# Autodesk Inventor assembly: Moving_Link_Fixation
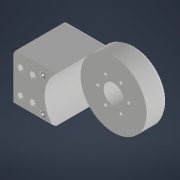
[picture p0: Inventor's stored thumbnail of the model, 180x180]
Saved by Autodesk Inventor 2021 (Build 250183000, 183)
## iProperties
Created: 2025-04-04
Part Number: Moving_Link_Fixation
Document SubType Name: Assembly
Designer: rocke
Author: rocke
## Documents named in this file (5)
- C:\Users\rocke\Documents\Robot Arm IPT\Moving Link Fixation\Moving_Link_Fixation.iam
- C:\Users\rocke\Documents\Inventor\Content Center Files\R2021\en-US\ISO 4032(2)\ISO 4032 - M4 - ISO.ipt
- C:\Users\rocke\Documents\Inventor\Content Center Files\R2021\en-US\ANSI B18.3.1M(1)\ANSI B18.3.1M - M4x0.7 x 65(2).ipt
- C:\Users\rocke\Documents\Robot Arm IPT\Moving Link Fixation\Moving_Link_Fixation_Small.ipt
- C:\Users\rocke\Documents\Robot Arm IPT\Moving Link Fixation\Moving_Link_Fixation_Large.ipt
## Components (6 placed, 4 different names)
1. Moving_Link_Fixation_Small:1 — Insert:1, Mate:5, Mate:6, Mate:7, Mate:9, Mate:10, Mate:11
2. Moving_Link_Fixation_Large:1 — Insert:1, Mate:8, Mate:12
3. Broached Socket Head Cap Screw - Metric M4x0.7 x 65:2 — Mate:9, Mate:10
4. ISO 4032 M4:1 — Mate:11, Mate:12
5. Broached Socket Head Cap Screw - Metric M4x0.7 x 65:1 — Mate:5, Mate:6
6. ISO 4032 M4:2 — Mate:7, Mate:8
## Relationships (9: Mate 8, Insert 1)
- Insert:1: Moving_Link_Fixation_Small:1 ↔ Moving_Link_Fixation_Large:1
- Mate:5: Moving_Link_Fixation_Small:1 ↔ Broached Socket Head Cap Screw - Metric M4x0.7 x 65:1
- Mate:6: Moving_Link_Fixation_Small:1 ↔ Broached Socket Head Cap Screw - Metric M4x0.7 x 65:1
- Mate:7: Moving_Link_Fixation_Small:1 ↔ ISO 4032 M4:2
- Mate:8: Moving_Link_Fixation_Large:1 ↔ ISO 4032 M4:2
- Mate:9: Moving_Link_Fixation_Small:1 ↔ Broached Socket Head Cap Screw - Metric M4x0.7 x 65:2
- Mate:10: Moving_Link_Fixation_Small:1 ↔ Broached Socket Head Cap Screw - Metric M4x0.7 x 65:2
- Mate:11: Moving_Link_Fixation_Small:1 ↔ ISO 4032 M4:1
- Mate:12: Moving_Link_Fixation_Large:1 ↔ ISO 4032 M4:1
